# Autodesk Inventor assembly: FinalAssembly
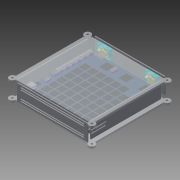
[picture p0: Inventor's stored thumbnail of the model, 180x180]
Saved by Autodesk Inventor 2015 (Build 190159000, 159)
## iProperties
Created: 2014-08-06
Part Number: FinalAssembly
Document SubType Name: Assembly
Designer: Patrick Camilleri
Author: Patrick Camilleri
## Documents named in this file (6)
- C:\Users\Patrick Camilleri\CAD\Test Box\FinalAssembly.iam
- C:\Users\Patrick Camilleri\CAD\Test Box\BasePlate.ipt
- C:\Users\Patrick Camilleri\CAD\Test Box\SidePanelFans.iam
- C:\Users\Patrick Camilleri\CAD\Test Box\Panel2.ipt
- C:\Users\Patrick Camilleri\CAD\Test Box\PanelFront.ipt
- C:\Users\Patrick Camilleri\CAD\Spin5 Board\Spin5 Inventor Simple 2\Imported Components\spin5v1_simple_2\spin5v1_simple_2.iam
## Components (7 placed, 5 different names)
1. Plate:1 — Flush:1
2. Plate:2
3. SidePanelFans:1 [sub-assembly]
4. Panel2:1
5. Panel2:2
6. PanelFront:1
7. spin5v1_simple_2:1 [sub-assembly]
## Relationships (1: Flush 1)
- Flush:1 (50 mm): Plate:1
